# Autodesk Inventor assembly: Assembly2
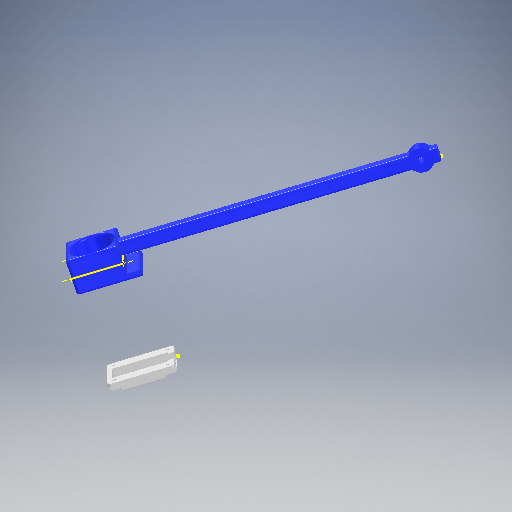
[picture p0: Inventor's stored thumbnail of the model, 512x512]
Saved by Autodesk Inventor 2025.3 (Build 293356000, 356)
## iProperties
Created: 2026-02-27
Part Number: Assembly2
Document SubType Name: Assembly
Designer: user
Mass: 65.9922 g
Surface Area: 166.08 cm^2
Volume: 40.3247 cm^3
Density: 1.63652 g/cm^3
Author: user
## Documents named in this file (3)
- C:\Ayman\Inventor Projects\Lifting Mechanism\Assembly2.iam
- C:\Ayman\Inventor Projects\Lifting Mechanism\arm.ipt
- C:\Ayman\Inventor Projects\Lifting Mechanism\final sensor housing.ipt
## Components (2 placed, 2 different names)
1. arm:1 — Mate:1, Mate:2, Mate:3, Mate:4
2. final sensor housing:1 — Mate:1, Mate:2, Mate:3, Mate:4
## Relationships (4: Mate 4)
- Mate:1: arm:1 ↔ final sensor housing:1
- Mate:2: arm:1 ↔ final sensor housing:1
- Mate:3: arm:1 ↔ final sensor housing:1
- Mate:4: arm:1 ↔ final sensor housing:1
